# Autodesk Inventor assembly: 022-DXP
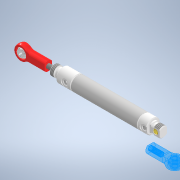
[picture p0: Inventor's stored thumbnail of the model, 180x180]
Saved by Autodesk Inventor 2022.3 (Build 263350000, 350)
## iProperties
Category: PARTsolutions
Company: BIMBA
Created: 2023-02-02
Part Number: 022-DXP
Catalog Web Link: www.cadenas.de
Description: Original Line Standard Air Cylinders-Standard Air Cylinders
Vendor: BIMBA
Document SubType Name: Assembly
Designer: psAdmin
Manufacturer: BIMBA
Mass: 15.3282 g
Surface Area: 156.05 cm^2
Volume: 15.3282 cm^3
Density: 1 g/cm^3
PSOL_IDENT_0: {$CADENAS_DATA/23d-libs/bimba/bimba_brand/bimba_imperial/bimba_full_line/original_line_cylinders/sta
PSOL_IDENT_1: ndard_air_cylinders/standard_air_cylinder_asmtab.prj},322 {VTYP=3D},{STYP=ASSTAB},{NB=022-DXP},{LINA=
PSOL_IDENT_2: 022-DXP},{NN=Original Line Standard Air Cylinders},{DATE=26.01.2023 11:48:58},{GEOMDATE=25.01.2023 0
PSOL_IDENT_3: 7:23:18},{VERSION=},{LINEID=40},{WBVAR=STROKE,ACTING,MNT,DER,NR,BM,CO,OO,VO,M,EE,EEL,K,Q,Y,G,T,HL,B,
PSOL_IDENT_4: H,SER,SR,NT,W,STPT1,STPT2,STPT3,STPT4,MB,PB,PRC,TB,MN},{WBNUMERIC=STROKE,EEL}  {NB=022-DXP},{LINA=02
PSOL_IDENT_5: 2-DXP},{KT=DUMMY},{PN=022-DXP},{PNC=022-DXP},{PNA=(NO ACCESSORIES)},{PNAHELP=},{DASH=-},{BORE1=0.562
PSOL_IDENT_6: 50000},{BORE=9/16\" (02)},{BOREPN=02},{STROKE=2.000},{STROKEALG=[0.011:50/0.001]},{STROKE1=2.000},{A
PSOL_IDENT_7: CTING=D},{ACTINGALG= '' , 'Single Acting' , 'R' , 'Reverse Single Acting (R)' , 'D' , 'Double Acting
PSOL_IDENT_8: (D)' },{ACTINGPN=D},{MNT=XP},{MNTALG= '' , 'Front Nose Mounting' , 'XP' , 'Double End or Rear Pivot
PSOL_IDENT_9: Mounting (XP)' , 'X' , 'Double End Mounting (X)' },{TYPE=},{MNTPN=XP},{DER=},{DERALG= '' , 'N/A' },
PSOL_IDENT_10: {NR=},{NRALG= '' , 'N/A' },{NRPN=},{BM=},{BMALG= '' , 'N/A' },{BMPN=},{CO=},{COALG= '' , 'N/A' },{OO=
PSOL_IDENT_11: },{OOALG= '', 'N/A' },{OOPN=},{VO=Z},{VOALG= 'Z' , 'N/A' },{VOPN=},{OOVOPN=},{M=},{MALG= '', 'Withou
PSOL_IDENT_12: t Magnet', 'M', 'With Magnet' },{EE=},{EEL=0.000},{EEMAX=48.0000},{EEALG= '', 'Without Extra Extensi
PSOL_IDENT_13: on', 'EE', 'With Extra Extension' },{EELALG=0},{EEPN=},{EEPN1=0.000},{K=},{KALG= '', 'Standard' , 'K'
PSOL_IDENT_14: , 'Ports Rotated 90deg K' },{KPN=},{Q=},{QALG= '' , 'N/A' },{QPN=},{Y=},{YALG= '' , 'With Pivot Bus
PSOL_IDENT_15: hing' },{YPN=},{YCON=Y},{F=},{FALG= '', 'Non-Coated (Standard)', 'F', 'Molycoated' },{FPN=},{G=},{GP
PSOL_IDENT_16: N=},{GPN99=},{T=},{TALG= '' , 'Standard -20° to 200°F (-29° to 95°C)' , 'N' , 'Low Temperature' , 'V'
PSOL_IDENT_17: , 'High Temperature' },{NPN=},{VPN=},{HL=},{HLALG= '' , 'Without Low Pressure Hydraulic' , 'HL' , '
PSOL_IDENT_18: With Low Pressure Hydraulic' },{B=},{BALG= '', 'W/out Bumpers' , 'B' , 'W/ Bumpers' },{BPN=},{H=},{H
PSOL_IDENT_19: ALG= '', 'N/A' },{HPN=},{SER=},{SERALG= '' , 'Without Spring Extend/Return' , 'JS' , 'With Spring Re
PSOL_IDENT_20: turn' , 'JR' , 'With Spring Extend' },{SR=},{SRALG= '' , 'Standard Stainless Steel' },{SRPN=},{SRCON=
PSOL_IDENT_21: 0},{NT=},{NTPN=},{W=},{WALG= '' , 'Without Wiper' , 'W' , 'With Wiper' },{WPN=},{E=},{EALG= '' , 'St
PSOL_IDENT_22: andard Seals/Lube' , 'E' , 'Non-Lube Seals/Lube' },{EPN=},{ST=},{STALG= '' , 'N/A' },{STPT1=},{STPT1
PSOL_IDENT_23: ALG= '' , 'N/A' },{STPT2=},{STPT2ALG= '' , 'N/A' },{STPT3=},{STPT3ALG= '' , 'N/A' },{STPT4=},{STPT4A
PSOL_IDENT_24: LG= '' , 'N/A' },{STPN=},{MB=},{MBALG= '' , 'Without Mounting Bracket' , 'F,D-770' , 'D-770 (front)'
PSOL_IDENT_25: , 'R,D-770' , 'D-770 (rear)' , '2x,D-770' , 'D-770 (front & rear)'},{MBPN=},{MBPNALL=D-770},{MBPNA
PSOL_IDENT_26: LLREAR=D-770},{PB=},{PBALG= '' , 'Without Pivot Bracket' , 'D-12321-A' , 'D-12321-A' },{PBPN=},{PBPN
PSOL_IDENT_27: ALL=D-12321-A},{PRC=},{PRCALG= '' , 'W/out Pivot Rod Clevis' , 'F,D-850' , 'D-850 (front)' },{PRCPN=
PSOL_IDENT_28: },{PRCPNALL=D-850},{TB=},{TBALG= '' , 'N/A' },{TBPN=},{TBPNALL=},{MN=},{MNALG= '' , 'N/A' },{MNPN=},
PSOL_IDENT_29: {MNCONF=},{MNCONR=},{TLEN=2.8870},{FRAC=7.5600},{RGCON=},{RGDACCON=R},{RHCON=P},{RHCON1=P},{RHCONON=
PSOL_IDENT_30: 1},{RHACCON=R},{FNUTCON=1},{RNUTCON=1},{FNUTPN=D-154},{RNUTPN=D-154},{FNUTTRANS=0.0000},{RNUTTRANS=0
PSOL_IDENT_31: .0000},{VHOLECON=0},{A1=1.1560},{A1N=1.0310},{A1P=1.1560},{A1B=0.0000},{A4=0.1570},{A4N=0.5310},{A4P=
PSOL_IDENT_32: 0.1570},{A5=0.0250},{A1H=0.969},{A1NH=0.5000},{A1PH=0.9690},{A1BH=0.0000},{A1SH=0.0000},{A2H=0.1570}
PSOL_IDENT_33: ,{A2NH=0.1570},{LENGTH=2.5600},{LENGTH1=2.5600},{LENGTH2=2.6100},{MUL=2.0000},{MUL11=2.0000},{MUL22=
PSOL_IDENT_34: 5.26},{MUL33=3.2600},{MUL2=2.0000},{MUL211=2.0000},{MUL222=2.6300},{MUL233=1.6300},{SSS=4.0000},{RGL
PSOL_IDENT_35: EN=1.0240},{RHLEN=0.6490},{SSS1=3.0000},{A13=0.7810},{DIF=0.0000},{G5=0.0000},{ON=0},{SSADD=0.0000},
PSOL_IDENT_36: {BADD=0.0000},{MADD=0.0000},{NVADD=0.0000},{TRACKL=2.5870},{TRACKCON=D-74168},{TRIMCON=0},{TRIMCON1=
PSOL_IDENT_37: 0},{PINCON=},{FSPACE=0.5104},{SPACE=0.0482},{TEXT=0.0844},{S1=0.0000},{D1=0.0000},{D1N=0.6150},{D1B=
PSOL_IDENT_38: 0.6150},{D1P=0.0000},{FA=0.690},{RA=0.6900},{PPATH=standard_air_cylinder_asmtpl.prj},{MATALGHTML=<b>
PSOL_IDENT_39: Standard Original Line:</b><dl><dt>Rod:</dt><dd>- Stainless Steel</dd><dd>&nbsp;&nbsp;(5/16 9/16 Bor
PSOL_IDENT_40: es)</dd><dd>- High Strength Carbon Steel</dd><dd>&nbsp;&nbsp;(3/4 3 Bore)</dd><dd>- Stainless Steel<
PSOL_IDENT_41: /dd><dd>&nbsp;&nbsp;(X style DXP/DX/DXDE)</dd><dt>Bearings:</dt><dd>- Sintered Bronze</dd><dt>Body:<
PSOL_IDENT_42: /dt><dd>- 304 Stainless Steel</dd><dt>End Caps:</dt><dd>- Aluminum</dd><dt>Seals:</dt><dd>- Buna N</
PSOL_IDENT_43: dd></dl>},{ASSCFGPRA=02DXP},{MBPNA=},{MNPNA=},{PRCPNA=},{ASSOPTACC=STPT4},{A=4.56},{HADD=0.0000},{WF
PSOL_IDENT_44: L=0},{QADD=0.000},{QADD1=0.030},{TEST=2.0000},{MNTB=},{STDNUTF=1},{STDNUTR=1},{STRK2D=0},{X2D=2},{ST
PSOL_IDENT_45: ROKESW=2.000},{EESW=0.000},{FCD=0},{BCD=0},{RCD=0},{CUSTADD=1.000},{FT=#10-32 UNF-2A},{FT1=#10-32 UN
PSOL_IDENT_46: F-2A},{FT2=7/16-20 UNF-2A},{PORT=UNF0.190},{PORT1=#10-32},{PORT2=UNF0.190},{FT11=7/16-20 UNF-2A},{FT
PSOL_IDENT_47: 12=7/16-20 UNF-2A},{B1=}
NB: 022-DXP
NN: Original Line Standard Air Cylinders
NT: Threaded (Standard)
NBSYN: $PNC.
LINA: 022-DXP
CATALOG: Bimba Products
PN: 022-DXP
PNA: (NO ACCESSORIES)
BORE: 9/16" (02)
STROKE: 2
ACTING: Double Acting (D)
MNT: Double End or Rear Pivot Mounting (XP)
DER: N/A
NR: N/A
CO: N/A
OO: N/A
VO: N/A
M: Without Magnet
EE: Without Extra Extension
EEL: 0
K: Standard
Q: N/A
Y: With Pivot Bushing
G: Standard Lube
T: Standard -20° to 200°F (-29° to 95°C)
HL: Without Low Pressure Hydraulic
B: W/out Bumpers
H: N/A
SER: Without Spring Extend/Return
SR: Standard Stainless Steel
W: Without Wiper
STPT1: N/A
STPT2: N/A
STPT3: N/A
STPT4: N/A
MB: Without Mounting Bracket
PB: Without Pivot Bracket
PRC: W/out Pivot Rod Clevis
TB: N/A
MN: N/A
A: 4.56
SUPPLIER: BIMBA
ARTICLENO: 022-DXP
BOMINFO: 022-DXP
CREATOR: CADENAS GmbH
Title: 022-DXP
Author: Cadenas PARTsolutions
Comments: Standard Air Cylinders
## Documents named in this file (8)
- C:\Users\mavericks\Desktop\2023-Charged-Up\COMMON PARTS\AIR CYLINDERS\BIMBA_022DXP (1)\AIS2022\022-DXP.iam
- C:\Users\mavericks\Desktop\2023-Charged-Up\COMMON PARTS\AIR CYLINDERS\BIMBA_022DXP (1)\AIS2022\022-DXP0000000_0_dummy.ipt
- C:\Users\mavericks\Desktop\2023-Charged-Up\COMMON PARTS\AIR CYLINDERS\BIMBA_022DXP (1)\AIS2022\02R000-0_rod_guide.ipt
- C:\Users\mavericks\Desktop\2023-Charged-Up\COMMON PARTS\AIR CYLINDERS\BIMBA_022DXP (1)\AIS2022\02R-2_8870.ipt
- C:\Users\mavericks\Desktop\2023-Charged-Up\COMMON PARTS\AIR CYLINDERS\BIMBA_022DXP (1)\AIS2022\02P0Y000_rear_head.ipt
- C:\Users\mavericks\Desktop\2023-Charged-Up\COMMON PARTS\AIR CYLINDERS\BIMBA_022DXP (1)\AIS2022\D-8597.ipt
- C:\Users\mavericks\Desktop\2023-Charged-Up\COMMON PARTS\AIR CYLINDERS\BIMBA_022DXP (1)\AIS2022\022-DXP0000_rod.ipt
- C:\Users\mavericks\Desktop\2023-Charged-Up\COMMON PARTS\AIR CYLINDERS\TieRod End\60685K311_PTFE-LINED ALUMINUM BALL JOINT ROD END.ipt
## Components (7 placed, 7 different names)
1. 022-DXP0000000_0_dummy:1
2. 02R000-0_rod_guide:1 — Mate:1, Mate:2
3. 02R-2_8870:1
4. 02P0Y000_rear_head:1 — Angle:1
5. D-8597:1
6. 022-DXP0000_rod:1 — Mate:1, Mate:2, Insert:1
7. 60685K311_PTFE-LINED ALUMINUM BALL JOINT ROD END:1 — Insert:1, Angle:1
## Relationships (4: Mate 2, Insert 1, Angle 1)
- Mate:1: 02R000-0_rod_guide:1 ↔ 022-DXP0000_rod:1
- Mate:2: 02R000-0_rod_guide:1 ↔ 022-DXP0000_rod:1
- Insert:1 (-6.35 mm): 022-DXP0000_rod:1 ↔ 60685K311_PTFE-LINED ALUMINUM BALL JOINT ROD END:1
- Angle:1 (0 deg): 02P0Y000_rear_head:1 ↔ 60685K311_PTFE-LINED ALUMINUM BALL JOINT ROD END:1
